# Autodesk Inventor assembly: Assembly2
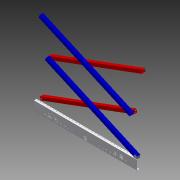
[picture p0: Inventor's stored thumbnail of the model, 180x180]
Saved by Autodesk Inventor 2015 (Build 190159000, 159)
## iProperties
Created: 2016-01-11
Part Number: Assembly2
Document SubType Name: Assembly
Designer: Applegate
Author: Applegate
## Documents named in this file (6)
- C:\Users\Applegate\Desktop\Chassy Files\Sissor Lift\Assembly2.iam
- C:\Users\Applegate\Desktop\Chassy Files\Sissor Lift\Long Bar.ipt
- C:\Users\Applegate\Desktop\Chassy Files\Sissor Lift\Gounded Clevis.ipt
- C:\Users\Applegate\Desktop\Chassy Files\Assembly\Imported Components\am-2951 AM14U2 Outside Sheet.ipt\am-2951 AM14U2 Outside Sheet.ipt.ipt
- C:\Users\Applegate\Desktop\Chassy Files\Sissor Lift\Long Bar Offset center.ipt
- am-2951 AM14U2 Outside Sheet.ipt
## Components (6 placed, 4 different names)
1. Gounded Clevis:1 — Rotational:2, Mate:1, Rotational:3
2. am-2951 AM14U2 Outside Sheet.ipt:1 — Rotational:2, Mate:1, Mate:2
3. Long Bar:1 — Rotational:3, Rotational:4, Rotational:6
4. Long Bar:2 — Rotational:5, Rotational:7
5. Long Bar Offset center:1 — Rotational:4, Mate:2, Rotational:5
6. Long Bar Offset center:2 — Rotational:6, Rotational:7
## Relationships (8: RevoluteJoint 6, Mate 2)
- Rotational:2 [RevoluteJoint]: Gounded Clevis:1 ↔ am-2951 AM14U2 Outside Sheet.ipt:1
- Mate:1: Gounded Clevis:1 ↔ am-2951 AM14U2 Outside Sheet.ipt:1
- Rotational:3 [RevoluteJoint]: Gounded Clevis:1 ↔ Long Bar:1
- Rotational:4 [RevoluteJoint]: Long Bar:1 ↔ Long Bar Offset center:1
- Mate:2: am-2951 AM14U2 Outside Sheet.ipt:1 ↔ Long Bar Offset center:1
- Rotational:5 [RevoluteJoint]: Long Bar:2 ↔ Long Bar Offset center:1
- Rotational:6 [RevoluteJoint]: Long Bar:1 ↔ Long Bar Offset center:2
- Rotational:7 [RevoluteJoint]: Long Bar:2 ↔ Long Bar Offset center:2
